# Autodesk Inventor assembly: ハンド
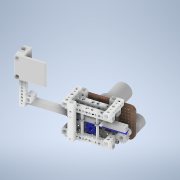
[picture p0: Inventor's stored thumbnail of the model, 180x180]
Saved by Autodesk Inventor 2020.3 (Build 243373000, 373)
## iProperties
Created: 2020-05-31
Part Number: ハンド
Document SubType Name: Assembly
Designer: totot
Mass: 321.88 g
Surface Area: 975.355 cm^2
Volume: 136.416 cm^3
Density: 2.35954 g/cm^3
Author: totot
## Documents named in this file (17)
- D:\mysvn\ロボコン\キャチロボ\キャチロボ設計図\ロボット\ハンド\ハンド.iam
- D:\mysvn\ロボコン\キャチロボ\キャチロボ設計図\ロボット\ハンド\ハンド9x9_1.ipt
- D:\mysvn\ロボコン\キャチロボ\キャチロボ設計図\ロボット\ハンド\ハンド9x9_2.ipt
- D:\mysvn\ロボコン\キャチロボ\キャチロボ設計図\ロボット\ハンド\ハンド9x9_3.ipt
- D:\mysvn\ロボコン\キャチロボ\キャチロボ設計図\ロボット\ハンド\ハンド_モータパネル.ipt
- D:\mysvn\ロボコン\キャチロボ\キャチロボ設計図\ロボット\ハンド\ハンド9x9_4.ipt
- D:\mysvn\ロボコン\キャチロボ\キャチロボ設計図\ロボット\ハンド\ハンド9x9_1_CPY.ipt
- D:\mysvn\ロボコン\キャチロボ\キャチロボ設計図\ロボット\ハンド\ハンド9x9_5.ipt
- D:\mysvn\ロボコン\キャチロボ\キャチロボ設計図\ロボット\ハンド\ハンド_ベアリングシャフト_1.ipt
- D:\mysvn\ロボコン\キャチロボ\キャチロボ設計図\ロボット\ハンド\ハンド_ベアリングシャフト_2.ipt
- D:\mysvn\ロボコン\キャチロボ\キャチロボ設計図\ロボット\ハンド\ハンド_ベアリング_4-8.ipt
- D:\mysvn\ロボコン\キャチロボ\キャチロボ設計図\ロボット\ハンド\ハンド9x9_6.ipt
- D:\mysvn\ロボコン\キャチロボ\キャチロボ設計図\ロボット\共有パーツ\RS_380.ipt
- D:\mysvn\ロボコン\キャチロボ\キャチロボ設計図\ロボット\共有パーツ\DR1-2000_On.ipt
- D:\mysvn\ロボコン\キャチロボ\キャチロボ設計図\ロボット\共有パーツ\PS1-15_On.ipt
- D:\mysvn\ロボコン\キャチロボ\キャチロボ設計図\ロボット\共有パーツ\ポテンションメーター_BI-7284.ipt
- D:\mysvn\ロボコン\キャチロボ\キャチロボ設計図\ロボット\共有パーツ\ハンド3D_L.ipt
## Components (33 placed, 16 different names)
1. ハンド9x9_1:1 — 挿入:4, 挿入:8, 挿入:15, 挿入:16, メイト:1, 正接:13
2. ハンド9x9_2:1 — 挿入:4, 挿入:5, 挿入:11, 挿入:22
3. ハンド9x9_3:1 — 挿入:5, 挿入:10, 挿入:16
4. ハンド9x9_3:2 — 挿入:7, 挿入:9, 挿入:15, 挿入:33, 挿入:34
5. ハンド9x9_2:2 — 挿入:7, 挿入:8, 挿入:14, 挿入:19
6. ハンド9x9_2:3 — 挿入:10, 挿入:12, 挿入:25
7. ハンド9x9_2:4 — 挿入:9, 挿入:13, 挿入:24
8. ハンド9x9_3:3 — 挿入:11, 挿入:12, 挿入:21, 挿入:26
9. ハンド9x9_3:4 — 挿入:13, 挿入:14, 挿入:20, 挿入:23, 挿入:32, 挿入:35
10. ハンド_モータパネル:1 — 挿入:45, 挿入:46, 挿入:47, 挿入:48, フラッシュ:10, 正接:16, メイト:6, 挿入:53, フラッシュ:16
11. ハンド9x9_4:1 — 挿入:19, 挿入:20, 挿入:21, 挿入:22, 挿入:46
12. ハンド9x9_4:2 — 挿入:23, 挿入:24, 挿入:25, 挿入:26, 挿入:45
13. ハンド9x9_1_CPY:1 — 挿入:31, 挿入:38, 挿入:51, 挿入:52
14. ハンド9x9_5:1 — 挿入:31, 挿入:39
15. ハンド_ベアリングシャフト_1:1 — 挿入:32, 正接:7
16. ハンド_ベアリングシャフト_1:2 — 挿入:33, 正接:12
17. ハンド_ベアリングシャフト_1:3 — 挿入:34, 正接:11
18. ハンド_ベアリングシャフト_1:4 — 挿入:35, 正接:8
19. ハンド_ベアリングシャフト_2:1 — 正接:3, 挿入:53
20. ハンド_ベアリングシャフト_2:2 — 正接:2, 正接:13, フラッシュ:10
21. ハンド_ベアリング_4-8:1 — 正接:2, メイト:1, フラッシュ:1, 正接:4
22. ハンド_ベアリング_4-8:2 — 正接:3, フラッシュ:1, 正接:5
23. ハンド9x9_6:1 — 挿入:38, 挿入:39, 正接:4, 正接:5, メイト:2, フラッシュ:2, フラッシュ:3, 正接:9, 正接:10, フラッシュ:5, フラッシュ:14, フラッシュ:16
24. RS_380:1 — 正接:6, 挿入:47, 挿入:48
25. DR1-2000_On:1 — メイト:2, フラッシュ:2, フラッシュ:3
26. PS1-15_On:1 — 正接:6, フラッシュ:15
27. ハンド_ベアリング_4-8:3 — 正接:8, 正接:10, フラッシュ:5, フラッシュ:6, フラッシュ:7, フラッシュ:8
28. ハンド_ベアリング_4-8:4 — 正接:7, 正接:9, フラッシュ:8
29. ハンド_ベアリング_4-8:5 — 正接:11, フラッシュ:6
30. ハンド_ベアリング_4-8:6 — フラッシュ:7, 正接:12
31. ポテンションメーター_BI-7284:1 — 正接:15, 正接:16, メイト:6
32. PS1-15_On:2 — 正接:15, フラッシュ:14, フラッシュ:15
33. ハンド3D_L:1 — 挿入:51, 挿入:52
## Relationships (62: Insert 34, Tangent 14, Flush 11, Mate 3)
- 挿入:4 [Insert]: ハンド9x9_1:1 ↔ ハンド9x9_2:1
- 挿入:5 [Insert]: ハンド9x9_2:1 ↔ ハンド9x9_3:1
- 挿入:7 [Insert]: ハンド9x9_3:2 ↔ ハンド9x9_2:2
- 挿入:8 [Insert]: ハンド9x9_1:1 ↔ ハンド9x9_2:2
- 挿入:9 [Insert]: ハンド9x9_3:2 ↔ ハンド9x9_2:4
- 挿入:10 [Insert]: ハンド9x9_3:1 ↔ ハンド9x9_2:3
- 挿入:11 [Insert]: ハンド9x9_2:1 ↔ ハンド9x9_3:3
- 挿入:12 [Insert]: ハンド9x9_2:3 ↔ ハンド9x9_3:3
- 挿入:13 [Insert]: ハンド9x9_2:4 ↔ ハンド9x9_3:4
- 挿入:14 [Insert]: ハンド9x9_2:2 ↔ ハンド9x9_3:4
- 挿入:15 [Insert]: ハンド9x9_1:1 ↔ ハンド9x9_3:2
- 挿入:16 [Insert]: ハンド9x9_1:1 ↔ ハンド9x9_3:1
- 挿入:19 [Insert]: ハンド9x9_2:2 ↔ ハンド9x9_4:1
- 挿入:20 [Insert]: ハンド9x9_3:4 ↔ ハンド9x9_4:1
- 挿入:21 [Insert]: ハンド9x9_3:3 ↔ ハンド9x9_4:1
- 挿入:22 [Insert]: ハンド9x9_2:1 ↔ ハンド9x9_4:1
- 挿入:23 [Insert]: ハンド9x9_3:4 ↔ ハンド9x9_4:2
- 挿入:24 [Insert]: ハンド9x9_2:4 ↔ ハンド9x9_4:2
- 挿入:25 [Insert]: ハンド9x9_2:3 ↔ ハンド9x9_4:2
- 挿入:26 [Insert]: ハンド9x9_3:3 ↔ ハンド9x9_4:2
- 挿入:31 [Insert]: ハンド9x9_1_CPY:1 ↔ ハンド9x9_5:1
- 挿入:32 [Insert]: ハンド9x9_3:4 ↔ ハンド_ベアリングシャフト_1:1
- 挿入:33 [Insert]: ハンド9x9_3:2 ↔ ハンド_ベアリングシャフト_1:2
- 挿入:34 [Insert]: ハンド9x9_3:2 ↔ ハンド_ベアリングシャフト_1:3
- 挿入:35 [Insert]: ハンド9x9_3:4 ↔ ハンド_ベアリングシャフト_1:4
- 正接:2 [Tangent]: ハンド_ベアリングシャフト_2:2 ↔ ハンド_ベアリング_4-8:1
- メイト:1 [Mate] (11.5 mm): ハンド9x9_1:1 ↔ ハンド_ベアリング_4-8:1
- 正接:3 [Tangent]: ハンド_ベアリングシャフト_2:1 ↔ ハンド_ベアリング_4-8:2
- フラッシュ:1 [Flush]: ハンド_ベアリング_4-8:1 ↔ ハンド_ベアリング_4-8:2
- 挿入:38 [Insert]: ハンド9x9_1_CPY:1 ↔ ハンド9x9_6:1
- 挿入:39 [Insert]: ハンド9x9_5:1 ↔ ハンド9x9_6:1
- 正接:4 [Tangent]: ハンド_ベアリング_4-8:1 ↔ ハンド9x9_6:1
- 正接:5 [Tangent]: ハンド_ベアリング_4-8:2 ↔ ハンド9x9_6:1
- メイト:2 [Mate]: ハンド9x9_6:1 ↔ DR1-2000_On:1
- フラッシュ:2 [Flush]: ハンド9x9_6:1 ↔ DR1-2000_On:1
- フラッシュ:3 [Flush] (0.5 mm): ハンド9x9_6:1 ↔ DR1-2000_On:1
- 正接:6 [Tangent]: RS_380:1 ↔ PS1-15_On:1
- 正接:7 [Tangent]: ハンド_ベアリングシャフト_1:1 ↔ ハンド_ベアリング_4-8:4
- 正接:8 [Tangent]: ハンド_ベアリングシャフト_1:4 ↔ ハンド_ベアリング_4-8:3
- 正接:9 [Tangent]: ハンド9x9_6:1 ↔ ハンド_ベアリング_4-8:4
- 正接:10 [Tangent]: ハンド9x9_6:1 ↔ ハンド_ベアリング_4-8:3
- フラッシュ:5 [Flush] (3 mm): ハンド9x9_6:1 ↔ ハンド_ベアリング_4-8:3
- 正接:11 [Tangent]: ハンド_ベアリングシャフト_1:3 ↔ ハンド_ベアリング_4-8:5
- フラッシュ:6 [Flush]: ハンド_ベアリング_4-8:3 ↔ ハンド_ベアリング_4-8:5
- フラッシュ:7 [Flush]: ハンド_ベアリング_4-8:3 ↔ ハンド_ベアリング_4-8:6
- 正接:12 [Tangent]: ハンド_ベアリングシャフト_1:2 ↔ ハンド_ベアリング_4-8:6
- フラッシュ:8 [Flush]: ハンド_ベアリング_4-8:3 ↔ ハンド_ベアリング_4-8:4
- 挿入:45 [Insert]: ハンド_モータパネル:1 ↔ ハンド9x9_4:2
- 挿入:46 [Insert]: ハンド_モータパネル:1 ↔ ハンド9x9_4:1
- 挿入:47 [Insert]: ハンド_モータパネル:1 ↔ RS_380:1
- 挿入:48 [Insert]: ハンド_モータパネル:1 ↔ RS_380:1
- 正接:13 [Tangent]: ハンド9x9_1:1 ↔ ハンド_ベアリングシャフト_2:2
- フラッシュ:10 [Flush]: ハンド_モータパネル:1 ↔ ハンド_ベアリングシャフト_2:2
- 正接:15 [Tangent]: ポテンションメーター_BI-7284:1 ↔ PS1-15_On:2
- 正接:16 [Tangent]: ハンド_モータパネル:1 ↔ ポテンションメーター_BI-7284:1
- メイト:6 [Mate]: ハンド_モータパネル:1 ↔ ポテンションメーター_BI-7284:1
- 挿入:51 [Insert]: ハンド9x9_1_CPY:1 ↔ ハンド3D_L:1
- 挿入:52 [Insert]: ハンド9x9_1_CPY:1 ↔ ハンド3D_L:1
- フラッシュ:14 [Flush] (-1 mm): ハンド9x9_6:1 ↔ PS1-15_On:2
- フラッシュ:15 [Flush]: PS1-15_On:1 ↔ PS1-15_On:2
- 挿入:53 [Insert]: ハンド_モータパネル:1 ↔ ハンド_ベアリングシャフト_2:1
- フラッシュ:16 [Flush]: ハンド_モータパネル:1 ↔ ハンド9x9_6:1
